# Autodesk Inventor assembly: latch
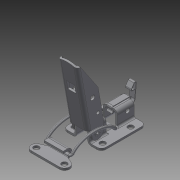
[picture p0: Inventor's stored thumbnail of the model, 180x180]
Saved by Autodesk Inventor 2015 (Build 190159000, 159)
## iProperties
Created: 2015-07-25
Part Number: latch
Document SubType Name: Assembly
Designer: Owner
Author: jim
Title: 1889A43.step
Description: STEP AP203
Creation Date: 2012-06-13
Sending System: SolidWorks 2009
Preprocessor: SwSTEP 2.0
Author: Owner
## Documents named in this file (7)
- C:\Users\Owner\Documents\GrabCAD\Driver Station\latch.iam
- C:\Users\Owner\Downloads\Imported Components\1889A430\TL_SECONDARY_CATCH_clf.ipt
- C:\Users\Owner\Downloads\Imported Components\1889A430\Imported.ipt
- C:\Users\Owner\Downloads\Imported Components\1889A430\TL_LOCKING_LEVER_clf.ipt
- C:\Users\Owner\Downloads\Imported Components\1889A430\TL_CURVED LINK_clf.ipt
- C:\Users\Owner\Downloads\Imported Components\1889A430\TL_LATCH_BASE_clf.ipt
- C:\Users\Owner\Downloads\Imported Components\1889A430\TL-17-201-52.ipt
## Components (6 placed, 6 different names)
1. TL_SECONDARY_CATCH_clf_1
2. Imported_2 — Mate:4, Mate:5, Mate:11
3. TL_LOCKING_LEVER_clf_3 — Mate:4, Mate:5, Mate:12
4. TL_CURVED LINK_clf_4 — Mate:10
5. TL_LATCH_BASE_clf_5 — Flush:1, Mate:11, Mate:12
6. TL-17-201-52_6 — Flush:1, Mate:10
## Relationships (6: Mate 5, Flush 1)
- Mate:4: Imported_2 ↔ TL_LOCKING_LEVER_clf_3
- Mate:5: Imported_2 ↔ TL_LOCKING_LEVER_clf_3
- Flush:1: TL_LATCH_BASE_clf_5 ↔ TL-17-201-52_6
- Mate:10: TL_CURVED LINK_clf_4 ↔ TL-17-201-52_6
- Mate:11: Imported_2 ↔ TL_LATCH_BASE_clf_5
- Mate:12: TL_LOCKING_LEVER_clf_3 ↔ TL_LATCH_BASE_clf_5
